# Autodesk Inventor assembly: UV
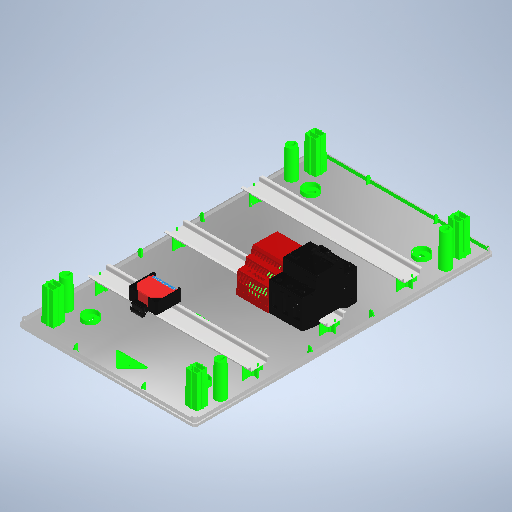
[picture p0: Inventor's stored thumbnail of the model, 512x512]
Saved by Autodesk Inventor 2025.1 (Build 291241000, 241)
## iProperties
Created: 2025-04-30
Part Number: UV
Document SubType Name: Assembly
Designer: jonah
Finish1_Appearance: Aluminum - Flat
Finish1_Area: 149457,263 mm^2
Author: jonah
## Documents named in this file (9)
- C:\Hauptspeicher\BZTG\ETS24\MC\005_Projekt_Kontrollpanel\Dokumentation\Installationszeichnung\UV.iam
- C:\Hauptspeicher\BZTG\ETS24\MC\005_Projekt_Kontrollpanel\Dokumentation\Installationszeichnung\N36-C\N36-C\N36-C.iam
- C:\Users\jonah\Downloads\1115669_KSTP1\1115669_KSTP1\1115669_KSTP1.ipt
- C:\Users\jonah\Downloads\1115669_KSTP1\5su13566kk10.ipt
- C:\Users\jonah\Downloads\1115669_KSTP1\5sl61166.ipt
- C:\Hauptspeicher\BZTG\ETS24\MC\005_Projekt_Kontrollpanel\Dokumentation\Installationszeichnung\shelly-1pm-1.snapshot.1\Shelly 1PM\Shelly 1PM\Shelly 1PM.ipt
- C:\Hauptspeicher\BZTG\ETS24\MC\005_Projekt_Kontrollpanel\Dokumentation\Installationszeichnung\shelly-1pm-1.snapshot.1\Shelly 1PM\SHWH_DIN_Klammer_V2.ipt
- C:\Hauptspeicher\BZTG\ETS24\MC\005_Projekt_Kontrollpanel\Dokumentation\Installationszeichnung\shelly-1pm-1.snapshot.1\Shelly 1PM\Shelly_plus-V1-A-WH.ipt
- C:\Hauptspeicher\BZTG\ETS24\MC\005_Projekt_Kontrollpanel\Dokumentation\Installationszeichnung\HDR-60\HDR-60\HDR-60.ipt
## Components (10 placed, 8 different names)
1. N36-C:1 [sub-assembly] — Passend:1, Passend:2, Passend:3, Passend:4, Passend:5
2. 1115669_KSTP1:1 — Passend:3, Winkel:1, Fluchtend:1, Fluchtend:2, Winkel:5
3. 1115669_KSTP1:2 — Passend:4, Winkel:1, Winkel:2, Fluchtend:1, Passend:15, Passend:16
4. 1115669_KSTP1:3 — Passend:5, Winkel:2, Winkel:3, Fluchtend:2, Winkel:4
5. 5su13566kk10:1 — Passend:13, Passend:14, Fluchtend:3, Fluchtend:4
6. 5sl61166:1 — Winkel:5, Passend:14, Fluchtend:3, Fluchtend:4
7. Shelly 1PM:1 — Passend:6, Passend:7, Passend:8
8. SHWH_DIN_Klammer_V2:1 — Passend:9, Passend:10, Passend:11, Passend:15, Passend:16
9. Shelly_plus-V1-A-WH:1 — Passend:6, Passend:7, Passend:8, Passend:9, Passend:10, Passend:11
10. HDR-60:1 — Winkel:4, Passend:13
## Relationships (24: Mate 15, Angle 5, Flush 4)
- Passend:1 [Mate]: N36-C:1
- Passend:2 [Mate]: N36-C:1
- Passend:3 [Mate]: N36-C:1 ↔ 1115669_KSTP1:1
- Passend:4 [Mate]: N36-C:1 ↔ 1115669_KSTP1:2
- Passend:5 [Mate]: N36-C:1 ↔ 1115669_KSTP1:3
- Winkel:1 [Angle] (0 deg): 1115669_KSTP1:1 ↔ 1115669_KSTP1:2
- Winkel:2 [Angle] (0 deg): 1115669_KSTP1:2 ↔ 1115669_KSTP1:3
- Winkel:3 [Angle] (90 deg): 1115669_KSTP1:3
- Fluchtend:1 [Flush]: 1115669_KSTP1:1 ↔ 1115669_KSTP1:2
- Fluchtend:2 [Flush]: 1115669_KSTP1:1 ↔ 1115669_KSTP1:3
- Passend:6 [Mate]: Shelly 1PM:1 ↔ Shelly_plus-V1-A-WH:1
- Passend:7 [Mate]: Shelly 1PM:1 ↔ Shelly_plus-V1-A-WH:1
- Passend:8 [Mate]: Shelly 1PM:1 ↔ Shelly_plus-V1-A-WH:1
- Passend:9 [Mate]: SHWH_DIN_Klammer_V2:1 ↔ Shelly_plus-V1-A-WH:1
- Passend:10 [Mate]: SHWH_DIN_Klammer_V2:1 ↔ Shelly_plus-V1-A-WH:1
- Passend:11 [Mate]: SHWH_DIN_Klammer_V2:1 ↔ Shelly_plus-V1-A-WH:1
- Winkel:4 [Angle] (0 deg): 1115669_KSTP1:3 ↔ HDR-60:1
- Passend:13 [Mate]: 5su13566kk10:1 ↔ HDR-60:1
- Winkel:5 [Angle] (0 deg): 1115669_KSTP1:1 ↔ 5sl61166:1
- Passend:14 [Mate]: 5su13566kk10:1 ↔ 5sl61166:1
- Fluchtend:3 [Flush]: 5su13566kk10:1 ↔ 5sl61166:1
- Fluchtend:4 [Flush]: 5su13566kk10:1 ↔ 5sl61166:1
- Passend:15 [Mate] (6 mm): 1115669_KSTP1:2 ↔ SHWH_DIN_Klammer_V2:1
- Passend:16 [Mate] (6 mm): 1115669_KSTP1:2 ↔ SHWH_DIN_Klammer_V2:1
## Named parameters: Finish1_Area = 1494.57, Finish2_Area = 20.4578
note: some values were not read from the file. Shown as the stored number, unit unknown: "Finish1_Area", "Finish2_Area".
